# Autodesk Inventor assembly: Configuration 1
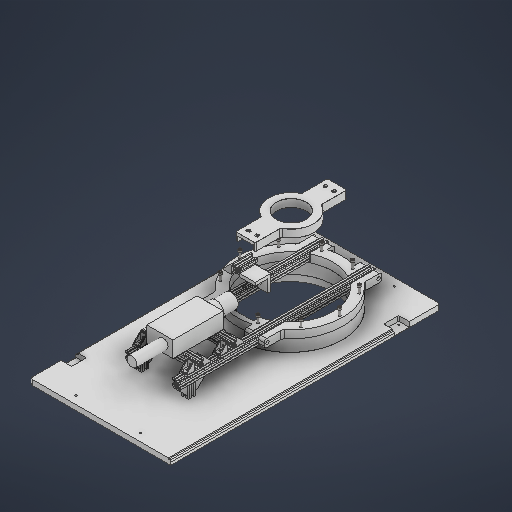
[picture p0: Inventor's stored thumbnail of the model, 512x512]
Saved by Autodesk Inventor 2025 (Build 290162000, 162)
## iProperties
Created: 2024-06-05
Part Number: Configuration 1
Document SubType Name: Assembly
Designer: AdminForWorker
Title: Printer Assembly v13
Author: AdminForWorker
## Documents named in this file (33)
- C:\Users\mayhe\OneDrive\Documents\GitHub\In-situ-monitoring-of-powder-bed-fusion-additive-manufacturing\system_development\Orichalcum\v0.2\Hardware_design\Full Printer Assembly\Printer Assembly.iam
- C:\Users\mayhe\OneDrive\Documents\GitHub\In-situ-monitoring-of-powder-bed-fusion-additive-manufacturing\system_development\Orichalcum\v0.2\Hardware_design\Full Printer Assembly\Printer Body v6.ipt
- C:\Users\mayhe\OneDrive\Documents\GitHub\In-situ-monitoring-of-powder-bed-fusion-additive-manufacturing\system_development\Orichalcum\v0.2\Hardware_design\Full Printer Assembly\Printer Frame.ipt
- C:\Users\mayhe\OneDrive\Documents\GitHub\In-situ-monitoring-of-powder-bed-fusion-additive-manufacturing\system_development\Orichalcum\v0.2\Hardware_design\Full Printer Assembly\overhead laser unit v1.ipt
- C:\Users\mayhe\OneDrive\Documents\GitHub\In-situ-monitoring-of-powder-bed-fusion-additive-manufacturing\system_development\Orichalcum\v0.2\Hardware_design\Full Printer Assembly\Part4.ipt
- C:\Users\mayhe\OneDrive\Documents\GitHub\In-situ-monitoring-of-powder-bed-fusion-additive-manufacturing\system_development\Orichalcum\v0.2\Hardware_design\custom-cover\cover\Updated Cover.ipt
- C:\Users\mayhe\OneDrive\Documents\GitHub\In-situ-monitoring-of-powder-bed-fusion-additive-manufacturing\system_development\Orichalcum\v0.2\Hardware_design\custom-cover\cylinder-parts\final-parts\Cylinder Bottom Ring.ipt
- C:\Users\mayhe\OneDrive\Documents\GitHub\In-situ-monitoring-of-powder-bed-fusion-additive-manufacturing\system_development\Orichalcum\v0.2\Hardware_design\custom-cover\cylinder-parts\final-parts\Cylinder Slidey Bit Housing.ipt
- C:\Users\mayhe\OneDrive\Documents\GitHub\In-situ-monitoring-of-powder-bed-fusion-additive-manufacturing\system_development\Orichalcum\v0.2\Hardware_design\custom-cover\cylinder-parts\Cylinder 80-20 Spacer_1.ipt
- C:\Users\mayhe\OneDrive\Documents\GitHub\In-situ-monitoring-of-powder-bed-fusion-additive-manufacturing\system_development\Orichalcum\v0.2\Hardware_design\custom-cover\cylinder-parts\Cylinder 80-20 Spacer_2.ipt
- C:\Users\mayhe\OneDrive\Documents\GitHub\In-situ-monitoring-of-powder-bed-fusion-additive-manufacturing\system_development\Orichalcum\v0.2\Hardware_design\custom-cover\cylinder-parts\cylinder-segments\Cylinder Segment .ipt
- C:\Users\mayhe\OneDrive\Documents\GitHub\In-situ-monitoring-of-powder-bed-fusion-additive-manufacturing\system_development\Orichalcum\v0.2\Hardware_design\custom-cover\cylinder-parts\final-parts\Cylinder Segment - 01.ipt
- C:\Users\mayhe\OneDrive\Documents\GitHub\In-situ-monitoring-of-powder-bed-fusion-additive-manufacturing\system_development\Orichalcum\v0.2\Hardware_design\custom-cover\cylinder-parts\cylinder-segments\Head Thing.ipt
- C:\Users\mayhe\OneDrive\Documents\GitHub\In-situ-monitoring-of-powder-bed-fusion-additive-manufacturing\system_development\Orichalcum\v0.2\Hardware_design\Full Printer Assembly\Plunger.ipt
- C:\Users\mayhe\OneDrive\Documents\GitHub\In-situ-monitoring-of-powder-bed-fusion-additive-manufacturing\system_development\Orichalcum\v0.2\Hardware_design\pzt-parts\PZT Assembly.iam
- C:\Users\mayhe\OneDrive\Documents\GitHub\In-situ-monitoring-of-powder-bed-fusion-additive-manufacturing\system_development\Orichalcum\v0.2\Hardware_design\Full Printer Assembly\Adapter Plate.ipt
- C:\Users\mayhe\OneDrive\Documents\GitHub\In-situ-monitoring-of-powder-bed-fusion-additive-manufacturing\system_development\Orichalcum\v0.2\Hardware_design\Full Printer Assembly\Build Plate.ipt
- C:\Users\mayhe\OneDrive\Documents\GitHub\In-situ-monitoring-of-powder-bed-fusion-additive-manufacturing\system_development\Orichalcum\v0.2\Hardware_design\Full Printer Assembly\Bottom Cap outlet.ipt
- C:\Users\mayhe\OneDrive\Documents\GitHub\In-situ-monitoring-of-powder-bed-fusion-additive-manufacturing\system_development\Orichalcum\v0.2\Hardware_design\pzt-parts\Capsule.ipt
- C:\Users\mayhe\OneDrive\Documents\GitHub\In-situ-monitoring-of-powder-bed-fusion-additive-manufacturing\system_development\Orichalcum\v0.2\Hardware_design\laser-vibrometer\Updated Laser Scanner.ipt
- C:\Users\mayhe\OneDrive\Documents\GitHub\In-situ-monitoring-of-powder-bed-fusion-additive-manufacturing\system_development\Orichalcum\v0.2\Hardware_design\custom-cover\8020-parts\20-2020-500-CL.ipt
- C:\Users\mayhe\OneDrive\Documents\GitHub\In-situ-monitoring-of-powder-bed-fusion-additive-manufacturing\system_development\Orichalcum\v0.2\Hardware_design\custom-cover\cylinder-parts\Cylinder 80-20 Spacer_1 Slant.ipt
- C:\Users\mayhe\OneDrive\Documents\GitHub\In-situ-monitoring-of-powder-bed-fusion-additive-manufacturing\system_development\Orichalcum\v0.2\Hardware_design\custom-cover\8020-parts\20-2020-140_25-CL.ipt
- C:\Users\mayhe\OneDrive\Documents\GitHub\In-situ-monitoring-of-powder-bed-fusion-additive-manufacturing\system_development\Orichalcum\v0.2\Hardware_design\custom-cover\8020-parts\20-2020-30-CL.ipt
- C:\Users\mayhe\OneDrive\Documents\GitHub\In-situ-monitoring-of-powder-bed-fusion-additive-manufacturing\system_development\Orichalcum\v0.2\Hardware_design\custom-cover\cover\Spacer Laser.ipt
- C:\Users\mayhe\OneDrive\Documents\GitHub\In-situ-monitoring-of-powder-bed-fusion-additive-manufacturing\system_development\Orichalcum\v0.2\Hardware_design\custom-cover\8020-parts\14056_m.ipt
- C:\Users\mayhe\OneDrive\Documents\Inventor\Content Center Files\R2025\en-US\ANSI B18.3.1M(6)\ANSI B18.3.1M - M5x0.8 x 80(1).ipt
- C:\Users\mayhe\OneDrive\Documents\GitHub\In-situ-monitoring-of-powder-bed-fusion-additive-manufacturing\system_development\Orichalcum\v0.2\Hardware_design\galvo-scanner\Other Galvo\Non-ThorLabs Galvo.ipt
- C:\Users\mayhe\OneDrive\Documents\GitHub\In-situ-monitoring-of-powder-bed-fusion-additive-manufacturing\system_development\Orichalcum\v0.2\Hardware_design\custom-cover\8020-parts\20-2020-41-CL.ipt
- C:\Users\mayhe\OneDrive\Documents\Inventor\Content Center Files\R2025\en-US\BS EN ISO 4762\BS EN ISO 4762 - M4 x 30(1).ipt
- C:\Users\mayhe\OneDrive\Documents\GitHub\In-situ-monitoring-of-powder-bed-fusion-additive-manufacturing\system_development\Orichalcum\v0.2\Hardware_design\custom-cover\8020-parts\13084_m.ipt
- C:\Users\mayhe\OneDrive\Documents\GitHub\In-situ-monitoring-of-powder-bed-fusion-additive-manufacturing\system_development\Orichalcum\v0.2\Hardware_design\custom-cover\cylinder-parts\cylinder-segments\Cylinder Segment - 10.ipt
- C:\Users\mayhe\OneDrive\Documents\GitHub\In-situ-monitoring-of-powder-bed-fusion-additive-manufacturing\system_development\Orichalcum\v0.2\Hardware_design\custom-cover\cylinder-parts\cylinder-segments\Cylinder Segment - Face.ipt
## Components (68 placed, 31 different names)
1. Printer Frame:1 — Flush:1, Mate:1, Mate:2, Mate:3, Flush:2, Flush:3, Rotational:5, Rotational:6, Angle:3, Angle:4
2. Printer Body v6:1 — Flush:1, Mate:1, Mate:2, Mate:5, Mate:6, Mate:7, Angle:2
3. overhead laser unit v1:1 — Mate:4, Angle:1, Flush:4
4. Part4:1 — Mate:3, Flush:2, Flush:3, Mate:4, Angle:1, Flush:4
5. Plunger:1 — Rotational:6
6. Plunger:2 — Rotational:5, Cylindrical:1, Rotational:9, Mate:68, Angle:2, Cylindrical:2
7. Bottom Cap outlet:1 — Rotational:9, Mate:68
8. Cylinder Segment - 10:2 — Cylindrical:4
9. Cylinder Segment - Face:3 — Cylindrical:4
10. Head Thing:1
11. Updated Cover:1 — Mate:5, Mate:6, Mate:7, Rotational:4, Mate:53
12. Build Plate:1 — Rotational:7, Rotational:8, Mate:67
13. Adapter Plate:1 — Rotational:7
14. PZT Assembly:1 [sub-assembly] — Rotational:8, Mate:67, Cylindrical:1, Angle:3
15. Capsule:1 — Rotational:10, Rotational:12, Mate:70
16. PZT Assembly:3 [sub-assembly] — Rotational:11, Cylindrical:2, Angle:4, Mate:69
17. Build Plate:3 — Rotational:10, Rotational:11, Mate:69, Mate:70
18. Adapter Plate:2 — Rotational:12
19. Non-ThorLabs Galvo:1 — Mate:113, Mate:114, Mate:115, Mate:117
20. 20-2020-41-CL:1 — Mate:113, Mate:114, Mate:116, Mate:119, Flush:31, Mate:120, Mate:121, Flush:32, Mate:122, Mate:123, Mate:124, Mate:125, Mate:132, Angle:5, Angle:6, Mate:137
21. BS EN ISO 4762 - Metric M4 x 30:1 — Mate:115, Mate:116
22. BS EN ISO 4762 - Metric M4 x 30:2 — Mate:117, Mate:119, Mate:137
23. 13084_m:1 — Flush:31, Mate:120, Mate:121, Mate:126
24. 13084_m:2 — Flush:32, Mate:122, Mate:123, Mate:127
25. 14056_m:15 — Mate:125, Mate:126, Mate:130, Mate:131, Angle:6
26. 14056_m:16 — Mate:124, Mate:127, Mate:128, Mate:129, Mate:132, Angle:5
27. 13084_m:3 — Mate:128, Mate:129, Mate:136
28. 13084_m:4 — Mate:130, Mate:131, Mate:133, Mate:134, Mate:135, Flush:33
29. Updated Laser Scanner:1 — Mate:76, Mate:77, Mate:79, Mate:80, Mate:81, Mate:82
30. 20-2020-140_25-CL:1 — Mate:79, Mate:80, Flush:12, Flush:14, Mate:89, Flush:19, Mate:91, Flush:20, Mate:97, Flush:23, Mate:99, Flush:24
31. 20-2020-140_25-CL:2 — Mate:81, Mate:82, Flush:16, Flush:18, Mate:93, Flush:21, Mate:95, Flush:22, Mate:101, Flush:25, Mate:103, Flush:26
32. 20-2020-30-CL:1 — Mate:83, Flush:7, Flush:8, Mate:106, Mate:112
33. 20-2020-30-CL:2 — Mate:84, Flush:9, Flush:10, Mate:108, Mate:110
34. Spacer Laser:1 — Mate:85, Flush:11, Flush:12, Mate:92, Mate:98
35. Spacer Laser:2 — Mate:86, Flush:13, Flush:14, Mate:90, Mate:100
36. Spacer Laser:3 — Mate:88, Flush:17, Flush:18, Mate:94, Mate:102
37. Spacer Laser:4 — Mate:87, Flush:15, Flush:16, Mate:96, Mate:104
38. 14056_m:1 — Mate:93, Mate:94, Flush:21
39. 14056_m:2 — Mate:95, Mate:96, Flush:22
40. 14056_m:3 — Mate:99, Mate:100, Flush:24
41. 14056_m:4 — Mate:101, Mate:102, Flush:25
42. 14056_m:5 — Mate:97, Mate:98, Flush:23
43. 14056_m:6 — Mate:103, Mate:104, Flush:26
44. 14056_m:7 — Mate:89, Mate:90, Flush:19
45. 14056_m:8 — Mate:91, Mate:92, Flush:20
46. 14056_m:9 — Mate:105, Mate:106, Flush:27
47. 14056_m:10 — Mate:107, Mate:108, Flush:28
48. 14056_m:12 — Mate:111, Mate:112, Flush:30
49. 14056_m:13 — Mate:109, Mate:110, Flush:29
50. 20-2020-500-CL:2 — Flush:5, Mate:72, Mate:73, Mate:83, Flush:7, Flush:8, Mate:85, Flush:11, Mate:87, Flush:15, Mate:105, Flush:27, Mate:111, Flush:30
51. 20-2020-500-CL:1 — Flush:6, Mate:74, Mate:75, Mate:84, Flush:9, Flush:10, Mate:86, Flush:13, Mate:88, Flush:17, Mate:107, Flush:28, Mate:109, Flush:29, Mate:133, Mate:134, Mate:135, Flush:33, Mate:136
52. Cylinder 80-20 Spacer_1 Slant:1 — Rotational:13, Mate:78
53. Cylinder 80-20 Spacer_2:1 — Mate:60, Mate:61, Mate:62, Mate:73
54. Cylinder 80-20 Spacer_2:2 — Mate:47, Mate:54, Mate:55, Mate:57, Flush:6, Mate:75
55. Cylinder 80-20 Spacer_1:3 — Mate:64, Mate:65, Mate:66, Flush:5
56. Cylinder Segment - 01:1 — Mate:47, Rotational:2, Mate:48, Rotational:13, Mate:78
57. Cylinder Slidey Bit Housing:1 — Rotational:2, Mate:48, Mate:76, Mate:77, Rotational:14, Rotational:15, Rotational:16, Rotational:17, Rotational:18, Rotational:19, Rotational:20, Rotational:21, Rotational:22, Rotational:23
58. Cylinder Bottom Ring:1 — Rotational:4, Mate:53, Mate:54, Mate:55, Mate:57, Mate:60, Mate:61, Mate:62, Mate:64, Mate:65, Mate:66, Mate:72, Mate:74
59. Forged Socket Head Cap Screw - Metric M5x0.8 x 80:1 — Rotational:23
60. Forged Socket Head Cap Screw - Metric M5x0.8 x 80:2 — Rotational:22
61. Forged Socket Head Cap Screw - Metric M5x0.8 x 80:4 — Rotational:21
62. Forged Socket Head Cap Screw - Metric M5x0.8 x 80:5 — Rotational:20
63. Forged Socket Head Cap Screw - Metric M5x0.8 x 80:6 — Rotational:19
64. Forged Socket Head Cap Screw - Metric M5x0.8 x 80:7 — Rotational:17
65. Forged Socket Head Cap Screw - Metric M5x0.8 x 80:8 — Rotational:15
66. Forged Socket Head Cap Screw - Metric M5x0.8 x 80:9 — Rotational:16
67. Forged Socket Head Cap Screw - Metric M5x0.8 x 80:10 — Rotational:14
68. Forged Socket Head Cap Screw - Metric M5x0.8 x 80:11 — Rotational:18
## Relationships (153: Mate 88, Flush 35, RevoluteJoint 21, Angle 6, CylindricalJoint 3)
- Flush:1: Printer Frame:1 ↔ Printer Body v6:1
- Mate:1: Printer Frame:1 ↔ Printer Body v6:1
- Mate:2 (92.5 mm): Printer Frame:1 ↔ Printer Body v6:1
- Mate:3: Printer Frame:1 ↔ Part4:1
- Flush:2 (28.5 mm): Printer Frame:1 ↔ Part4:1
- Flush:3 (-27 mm): Printer Frame:1 ↔ Part4:1
- Mate:4: overhead laser unit v1:1 ↔ Part4:1
- Angle:1 (179.9998 deg): overhead laser unit v1:1 ↔ Part4:1
- Flush:4 (-30 mm): overhead laser unit v1:1 ↔ Part4:1
- Mate:5: Printer Body v6:1 ↔ Updated Cover:1
- Mate:6: Printer Body v6:1 ↔ Updated Cover:1
- Mate:7: Printer Body v6:1 ↔ Updated Cover:1
- Mate:47: Cylinder 80-20 Spacer_2:2 ↔ Cylinder Segment - 01:1
- Rotational:2 [RevoluteJoint]: Cylinder Segment - 01:1 ↔ Cylinder Slidey Bit Housing:1
- Mate:48: Cylinder Segment - 01:1 ↔ Cylinder Slidey Bit Housing:1
- Rotational:4 [RevoluteJoint]: Updated Cover:1 ↔ Cylinder Bottom Ring:1
- Mate:53: Updated Cover:1 ↔ Cylinder Bottom Ring:1
- Mate:54: Cylinder 80-20 Spacer_2:2 ↔ Cylinder Bottom Ring:1
- Mate:55: Cylinder 80-20 Spacer_2:2 ↔ Cylinder Bottom Ring:1
- Mate:57: Cylinder 80-20 Spacer_2:2 ↔ Cylinder Bottom Ring:1
- Mate:60: Cylinder 80-20 Spacer_2:1 ↔ Cylinder Bottom Ring:1
- Mate:61: Cylinder 80-20 Spacer_2:1 ↔ Cylinder Bottom Ring:1
- Mate:62: Cylinder 80-20 Spacer_2:1 ↔ Cylinder Bottom Ring:1
- Mate:64: Cylinder 80-20 Spacer_1:3 ↔ Cylinder Bottom Ring:1
- Mate:65: Cylinder 80-20 Spacer_1:3 ↔ Cylinder Bottom Ring:1
- Mate:66: Cylinder 80-20 Spacer_1:3 ↔ Cylinder Bottom Ring:1
- Rotational:5 [RevoluteJoint]: Printer Frame:1 ↔ Plunger:2
- Rotational:6 [RevoluteJoint]: Printer Frame:1 ↔ Plunger:1
- Rotational:7 [RevoluteJoint]: Build Plate:1 ↔ Adapter Plate:1
- Rotational:8 [RevoluteJoint]: Build Plate:1 ↔ PZT Assembly:1
- Mate:67: Build Plate:1 ↔ PZT Assembly:1
- Cylindrical:1: Plunger:2 ↔ PZT Assembly:1
- Rotational:9 [RevoluteJoint]: Plunger:2 ↔ Bottom Cap outlet:1
- Mate:68: Plunger:2 ↔ Bottom Cap outlet:1
- Angle:2 (0 deg): Printer Body v6:1 ↔ Plunger:2
- Angle:3 (0 deg): Printer Frame:1 ↔ PZT Assembly:1
- Rotational:10 [RevoluteJoint]: Capsule:1 ↔ Build Plate:3
- Rotational:11 [RevoluteJoint]: PZT Assembly:3 ↔ Build Plate:3
- Rotational:12 [RevoluteJoint]: Capsule:1 ↔ Adapter Plate:2
- Cylindrical:2: Plunger:2 ↔ PZT Assembly:3
- Angle:4 (0 deg): Printer Frame:1 ↔ PZT Assembly:3
- Mate:69: PZT Assembly:3 ↔ Build Plate:3
- Mate:70: Capsule:1 ↔ Build Plate:3
- Flush:5: 20-2020-500-CL:2 ↔ Cylinder 80-20 Spacer_1:3
- Mate:72: 20-2020-500-CL:2 ↔ Cylinder Bottom Ring:1
- Mate:73: 20-2020-500-CL:2 ↔ Cylinder 80-20 Spacer_2:1
- Flush:6: 20-2020-500-CL:1 ↔ Cylinder 80-20 Spacer_2:2
- Mate:74: 20-2020-500-CL:1 ↔ Cylinder Bottom Ring:1
- Mate:75: 20-2020-500-CL:1 ↔ Cylinder 80-20 Spacer_2:2
- Mate:76 (-15 mm): Updated Laser Scanner:1 ↔ Cylinder Slidey Bit Housing:1
- Mate:77: Updated Laser Scanner:1 ↔ Cylinder Slidey Bit Housing:1
- Rotational:13 [RevoluteJoint]: Cylinder 80-20 Spacer_1 Slant:1 ↔ Cylinder Segment - 01:1
- Mate:78: Cylinder 80-20 Spacer_1 Slant:1 ↔ Cylinder Segment - 01:1
- Mate:79: Updated Laser Scanner:1 ↔ 20-2020-140_25-CL:1
- Mate:80: Updated Laser Scanner:1 ↔ 20-2020-140_25-CL:1
- Mate:81: Updated Laser Scanner:1 ↔ 20-2020-140_25-CL:2
- Mate:82: Updated Laser Scanner:1 ↔ 20-2020-140_25-CL:2
- Mate:83: 20-2020-30-CL:1 ↔ 20-2020-500-CL:2
- Flush:7: 20-2020-30-CL:1 ↔ 20-2020-500-CL:2
- Flush:8 (20 mm): 20-2020-30-CL:1 ↔ 20-2020-500-CL:2
- Mate:84: 20-2020-30-CL:2 ↔ 20-2020-500-CL:1
- Flush:9: 20-2020-30-CL:2 ↔ 20-2020-500-CL:1
- Flush:10 (20 mm): 20-2020-30-CL:2 ↔ 20-2020-500-CL:1
- Mate:85: Spacer Laser:1 ↔ 20-2020-500-CL:2
- Flush:11: Spacer Laser:1 ↔ 20-2020-500-CL:2
- Flush:12 (-20 mm): 20-2020-140_25-CL:1 ↔ Spacer Laser:1
- Mate:86: Spacer Laser:2 ↔ 20-2020-500-CL:1
- Flush:13: Spacer Laser:2 ↔ 20-2020-500-CL:1
- Flush:14 (-20 mm): 20-2020-140_25-CL:1 ↔ Spacer Laser:2
- Mate:87: Spacer Laser:4 ↔ 20-2020-500-CL:2
- Flush:15: Spacer Laser:4 ↔ 20-2020-500-CL:2
- Flush:16 (-20 mm): 20-2020-140_25-CL:2 ↔ Spacer Laser:4
- Mate:88: Spacer Laser:3 ↔ 20-2020-500-CL:1
- Flush:17: Spacer Laser:3 ↔ 20-2020-500-CL:1
- Flush:18 (-20 mm): 20-2020-140_25-CL:2 ↔ Spacer Laser:3
- Mate:89: 20-2020-140_25-CL:1 ↔ 14056_m:7
- Mate:90: Spacer Laser:2 ↔ 14056_m:7
- Flush:19 (1.5 mm): 20-2020-140_25-CL:1 ↔ 14056_m:7
- Mate:91: 20-2020-140_25-CL:1 ↔ 14056_m:8
- Mate:92: Spacer Laser:1 ↔ 14056_m:8
- Flush:20 (1.5 mm): 20-2020-140_25-CL:1 ↔ 14056_m:8
- Mate:93: 20-2020-140_25-CL:2 ↔ 14056_m:1
- Mate:94: Spacer Laser:3 ↔ 14056_m:1
- Flush:21 (1.5 mm): 20-2020-140_25-CL:2 ↔ 14056_m:1
- Mate:95: 20-2020-140_25-CL:2 ↔ 14056_m:2
- Mate:96: Spacer Laser:4 ↔ 14056_m:2
- Flush:22 (1.5 mm): 20-2020-140_25-CL:2 ↔ 14056_m:2
- Mate:97: 20-2020-140_25-CL:1 ↔ 14056_m:5
- Mate:98: Spacer Laser:1 ↔ 14056_m:5
- Flush:23 (1.5 mm): 20-2020-140_25-CL:1 ↔ 14056_m:5
- Mate:99: 20-2020-140_25-CL:1 ↔ 14056_m:3
- Mate:100: Spacer Laser:2 ↔ 14056_m:3
- Flush:24 (1.5 mm): 20-2020-140_25-CL:1 ↔ 14056_m:3
- Mate:101: 20-2020-140_25-CL:2 ↔ 14056_m:4
- Mate:102: Spacer Laser:3 ↔ 14056_m:4
- Flush:25 (1.5 mm): 20-2020-140_25-CL:2 ↔ 14056_m:4
- Mate:103: 20-2020-140_25-CL:2 ↔ 14056_m:6
- Mate:104: Spacer Laser:4 ↔ 14056_m:6
- Flush:26 (1.5 mm): 20-2020-140_25-CL:2 ↔ 14056_m:6
- Mate:105: 14056_m:9 ↔ 20-2020-500-CL:2
- Mate:106: 20-2020-30-CL:1 ↔ 14056_m:9
- Flush:27 (1.5 mm): 14056_m:9 ↔ 20-2020-500-CL:2
- Mate:107: 14056_m:10 ↔ 20-2020-500-CL:1
- Mate:108: 20-2020-30-CL:2 ↔ 14056_m:10
- Flush:28 (1.5 mm): 14056_m:10 ↔ 20-2020-500-CL:1
- Mate:109: 14056_m:13 ↔ 20-2020-500-CL:1
- Mate:110: 20-2020-30-CL:2 ↔ 14056_m:13
- Flush:29 (1.5 mm): 14056_m:13 ↔ 20-2020-500-CL:1
- Mate:111: 14056_m:12 ↔ 20-2020-500-CL:2
- Mate:112: 20-2020-30-CL:1 ↔ 14056_m:12
- Flush:30 (1.5 mm): 14056_m:12 ↔ 20-2020-500-CL:2
- Rotational:14 [RevoluteJoint]: Cylinder Slidey Bit Housing:1 ↔ Forged Socket Head Cap Screw - Metric M5x0.8 x 80:10
- Rotational:15 [RevoluteJoint]: Cylinder Slidey Bit Housing:1 ↔ Forged Socket Head Cap Screw - Metric M5x0.8 x 80:8
- Rotational:16 [RevoluteJoint]: Cylinder Slidey Bit Housing:1 ↔ Forged Socket Head Cap Screw - Metric M5x0.8 x 80:9
- Rotational:17 [RevoluteJoint]: Cylinder Slidey Bit Housing:1 ↔ Forged Socket Head Cap Screw - Metric M5x0.8 x 80:7
- Rotational:18 [RevoluteJoint]: Cylinder Slidey Bit Housing:1 ↔ Forged Socket Head Cap Screw - Metric M5x0.8 x 80:11
- Rotational:19 [RevoluteJoint]: Cylinder Slidey Bit Housing:1 ↔ Forged Socket Head Cap Screw - Metric M5x0.8 x 80:6
- Rotational:20 [RevoluteJoint]: Cylinder Slidey Bit Housing:1 ↔ Forged Socket Head Cap Screw - Metric M5x0.8 x 80:5
- Rotational:21 [RevoluteJoint]: Cylinder Slidey Bit Housing:1 ↔ Forged Socket Head Cap Screw - Metric M5x0.8 x 80:4
- Rotational:22 [RevoluteJoint]: Cylinder Slidey Bit Housing:1 ↔ Forged Socket Head Cap Screw - Metric M5x0.8 x 80:2
- Rotational:23 [RevoluteJoint]: Cylinder Slidey Bit Housing:1 ↔ Forged Socket Head Cap Screw - Metric M5x0.8 x 80:1
- Mate:113 (4 mm): Non-ThorLabs Galvo:1 ↔ 20-2020-41-CL:1
- Mate:114: Non-ThorLabs Galvo:1 ↔ 20-2020-41-CL:1
- Mate:115: Non-ThorLabs Galvo:1 ↔ BS EN ISO 4762 - Metric M4 x 30:1
- Mate:116: 20-2020-41-CL:1 ↔ BS EN ISO 4762 - Metric M4 x 30:1
- Mate:117: Non-ThorLabs Galvo:1 ↔ BS EN ISO 4762 - Metric M4 x 30:2
- Mate:119: 20-2020-41-CL:1 ↔ BS EN ISO 4762 - Metric M4 x 30:2
- Flush:31 (-1.1 mm): 20-2020-41-CL:1 ↔ 13084_m:1
- Mate:120: 20-2020-41-CL:1 ↔ 13084_m:1
- Mate:121 (0.15 mm): 20-2020-41-CL:1 ↔ 13084_m:1
- Flush:32 (-1.1 mm): 20-2020-41-CL:1 ↔ 13084_m:2
- Mate:122: 20-2020-41-CL:1 ↔ 13084_m:2
- Mate:123 (0.15 mm): 20-2020-41-CL:1 ↔ 13084_m:2
- Mate:124: 20-2020-41-CL:1 ↔ 14056_m:16
- Mate:125: 20-2020-41-CL:1 ↔ 14056_m:15
- Mate:126: 13084_m:1 ↔ 14056_m:15
- Mate:127: 13084_m:2 ↔ 14056_m:16
- Mate:128 (55 mm): 14056_m:16 ↔ 13084_m:3
- Mate:129: 14056_m:16 ↔ 13084_m:3
- Mate:130 (55 mm): 14056_m:15 ↔ 13084_m:4
- Mate:131: 14056_m:15 ↔ 13084_m:4
- Mate:132: 20-2020-41-CL:1 ↔ 14056_m:16
- Angle:5 (0 deg): 20-2020-41-CL:1 ↔ 14056_m:16
- Angle:6 (0 deg): 20-2020-41-CL:1 ↔ 14056_m:15
- Mate:133: 13084_m:4 ↔ 20-2020-500-CL:1
- Mate:134: 13084_m:4 ↔ 20-2020-500-CL:1
- Mate:135 (0.15 mm): 13084_m:4 ↔ 20-2020-500-CL:1
- Flush:33 (240 mm): 13084_m:4 ↔ 20-2020-500-CL:1
- Cylindrical:4: Cylinder Segment - 10:2 ↔ Cylinder Segment - Face:3
- Mate:136 (0.11 mm): 13084_m:3 ↔ 20-2020-500-CL:1
- Mate:137: 20-2020-41-CL:1 ↔ BS EN ISO 4762 - Metric M4 x 30:2
- Flush:34 (382.875 mm)
- Flush:35 (465.042 mm)
